# Autodesk Inventor assembly: BRZ-A200
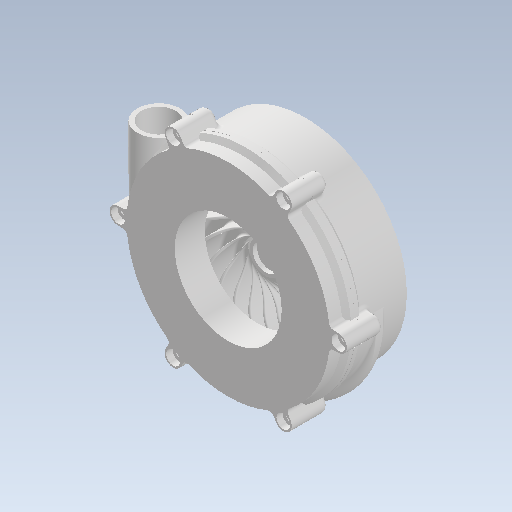
[picture p0: Inventor's stored thumbnail of the model, 512x512]
Saved by Autodesk Inventor 2020 (Build 240168000, 168)
## iProperties
Created: 2020-04-09
Part Number: BRZ-A200
Document SubType Name: Assembly
Designer: John K
Author: John K
## Documents named in this file (5)
- \\Mac\Home\Desktop\3D\Breeze thing\Breeze V2\Impeller Assembly\BRZ-A200.iam
- \\Mac\Home\Desktop\3D\Breeze thing\Breeze V2\Impeller Assembly\BRZ-P202.ipt
- \\Mac\Home\Desktop\3D\Breeze thing\Breeze V2\Impeller Assembly\BRZ-P201.ipt
- \\Mac\Home\Desktop\3D\Breeze thing\Breeze V2\Impeller Assembly\BRZ-P203.ipt
- \\Mac\Home\Desktop\3D\Breeze thing\Breeze V2\Impeller Assembly\Commercial Parts\McMaster\93mm O-Ring 1302N088.ipt
## Components (4 placed, 4 different names)
1. BRZ-P202:1 — Mate:1, Mate:2, Insert:1, Mate:3
2. BRZ-P201:1 — Mate:1, Mate:2
3. BRZ-P203:1 — Insert:1
4. 93mm O-Ring 1302N088:1 — Mate:3
## Relationships (4: Mate 3, Insert 1)
- Mate:1: BRZ-P202:1 ↔ BRZ-P201:1
- Mate:2 (2.5 mm): BRZ-P202:1 ↔ BRZ-P201:1
- Insert:1: BRZ-P202:1 ↔ BRZ-P203:1
- Mate:3: BRZ-P202:1 ↔ 93mm O-Ring 1302N088:1
